# Autodesk Inventor assembly: Firing Pin
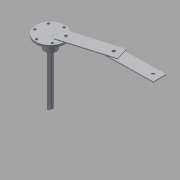
[picture p0: Inventor's stored thumbnail of the model, 180x180]
Saved by Autodesk Inventor 2013 (Build 170138000, 138)
## iProperties
Created: 2013-01-27
Part Number: Firing Pin
Document SubType Name: Assembly
Designer: carneeki
Author: carneeki
## Documents named in this file (5)
- C:\Autodesk\gruntmaster6000-cad\Shooter6000-cad\Shooter\Firing Pin\Firing Pin.iam
- C:\Autodesk\gruntmaster6000-cad\Shooter6000-cad\Shooter\Firing Pin\Part4.ipt
- C:\Autodesk\gruntmaster6000-cad\Shooter6000-cad\Shooter\Firing Pin\10mm-key-hub-am-0985.ipt
- C:\Autodesk\gruntmaster6000-cad\Shooter6000-cad\Shooter\Firing Pin\PG-Gearmotor-Shaft.ipt
- C:\Autodesk\gruntmaster6000-cad\Shooter6000-cad\Shooter\Firing Pin\Theta Bar.ipt
## Components (5 placed, 5 different names)
1. PG-Gearmotor-Shaft:1 — Flush:1, Mate:2, Mate:4, Mate:7
2. Ram — Insert:2, Mate:6
3. 10mm-key-hub-am-0985:1 — Flush:1, Mate:2, Insert:1, Mate:7
4. Z Bar — Mate:5, Insert:1, Insert:2
5. Mount Bar — Mate:4, Mate:5, Mate:6
## Relationships (8: Mate 5, Insert 2, Flush 1)
- Flush:1: PG-Gearmotor-Shaft:1 ↔ 10mm-key-hub-am-0985:1
- Mate:2: PG-Gearmotor-Shaft:1 ↔ 10mm-key-hub-am-0985:1
- Mate:4: PG-Gearmotor-Shaft:1 ↔ Mount Bar
- Mate:5: Z Bar ↔ Mount Bar
- Insert:1: 10mm-key-hub-am-0985:1 ↔ Z Bar
- Insert:2: Ram ↔ Z Bar
- Mate:6: Ram ↔ Mount Bar
- Mate:7: PG-Gearmotor-Shaft:1 ↔ 10mm-key-hub-am-0985:1
